# Autodesk Inventor assembly: Leg_joint_roll_pitch
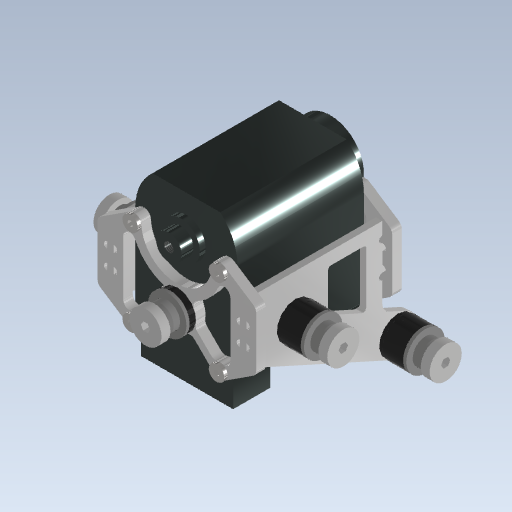
[picture p0: Inventor's stored thumbnail of the model, 512x512]
Saved by Autodesk Inventor 2020 (Build 240168000, 168)
## iProperties
Part Number: Leg_joint_roll_pitch
Document SubType Name: Assembly
Designer: Masato Kubotera
Mass: 155.537 g
Surface Area: 333.044 cm^2
Volume: 75.5065 cm^3
Density: 2.05992 g/cm^3
Author: Masato Kubotera
## Documents named in this file (16)
- C:\Users\Masato\Documents\Inventor\CIT Brains_Inventor\OpenPlatform_ver3_0 - Ver4_1branch\LowerBody\Leg_joit\Leg_joint_roll_pitch.iam
- C:\Users\Masato\Documents\Inventor\CIT Brains_Inventor\OpenPlatform_ver3_0 - Ver4_1branch\LowerBody\Leg_joit\Leg_joint_pitch_frame.ipt
- C:\Users\Masato\Documents\Inventor\CIT Brains_Inventor\OpenPlatform_ver3_0 - Ver4_1branch\LowerBody\Leg_joit\Leg_joint_roll_frame.ipt
- C:\Users\Masato\Documents\Inventor\CIT Brains_Inventor\OpenPlatform_ver3_0\Ready_Made\B3M11xx.ipt
- C:\Users\Masato\Documents\Inventor\CIT Brains_Inventor\OpenPlatform_ver3_0 - Ver4_1branch\Ready_Made\Screw\M2_6-20.ipt
- C:\Users\Masato\Documents\Inventor\CIT Brains_Inventor\OpenPlatform_ver3_0 - Ver4_1branch\Ready_Made\Screw\M2_6-15.ipt
- C:\Users\Masato\Documents\Inventor\CIT Brains_Inventor\OpenPlatform_ver3_0\Ready_Made\80F-0603.ipt
- C:\Users\Masato\Documents\Inventor\CIT Brains_Inventor\OpenPlatform_ver3_0\Ready_Made\CC-0612-15B.ipt
- C:\Users\Masato\Documents\Inventor\CIT Brains_Inventor\OpenPlatform_ver3_0\Ready_Made\CC-0612-50B.ipt
- C:\Users\Masato\Documents\Inventor\CIT Brains_Inventor\OpenPlatform_ver3_0 - Ver4_1branch\Ready_Made\SF419.ipt
- C:\Users\Masato\Documents\Inventor\CIT Brains_Inventor\OpenPlatform_ver3_0 - Ver4_1branch\Ready_Made\UUW-0412-10BH.ipt
- C:\Users\Masato\Documents\Inventor\CIT Brains_Inventor\OpenPlatform_ver3_0 - Ver4_1branch\Ready_Made\SLSBF6-39_5-M4-N4.ipt
- C:\Users\Masato\Documents\Inventor\CIT Brains_Inventor\OpenPlatform_ver3_0 - Ver4_1branch\Ready_Made\DBTS4-11-6.ipt
- C:\Users\Masato\Documents\Inventor\CIT Brains_Inventor\OpenPlatform_ver3_0 - Ver4_1branch\Ready_Made\DBS4-5-5.ipt
- C:\Users\Masato\Documents\Inventor\CIT Brains_Inventor\OpenPlatform_ver3_0 - Ver4_1branch\Ready_Made\DBTS4-10-4.ipt
- C:\Users\Masato\Documents\Inventor\CIT Brains_Inventor\OpenPlatform_ver3_0 - Ver4_1branch\Ready_Made\S4-07-3W.ipt
## Components (47 placed, 15 different names)
1. Leg_joint_pitch_frame:1 — フラッシュ:1, 挿入:192, 挿入:197, メイト:13
2. Leg_joint_pitch_frame:2 — フラッシュ:1, メイト:11, メイト:12, フラッシュ:7, 挿入:193, 挿入:194, 挿入:198
3. B3M11xx:1 — フラッシュ:6, メイト:8, メイト:10, 挿入:152, 挿入:153, 挿入:154, 挿入:155, 挿入:180, 挿入:181, 挿入:182, 挿入:183
4. M2_6-20:1 — 挿入:157
5. M2_6-20:2 — 挿入:159
6. M2_6-20:3 — 挿入:158
7. M2_6-20:4 — 挿入:160
8. M2_6-15:2 — 挿入:185
9. M2_6-15:3 — 挿入:186
10. 80F-0603:1 — 挿入:214
11. 80F-0603:3 — 挿入:130
12. 80F-0603:4 — 挿入:131
13. 80F-0603:5 — 挿入:129
14. 80F-0603:6 — 挿入:128
15. CC-0612-15B:1 — 挿入:114, 挿入:199
16. CC-0612-15B:2 — 挿入:115, 挿入:200
17. CC-0612-15B:3 — 挿入:116, 挿入:201
18. CC-0612-15B:4 — 挿入:117, 挿入:202
19. CC-0612-50B:1 — 挿入:114, 挿入:130
20. CC-0612-50B:2 — 挿入:115, 挿入:131
21. CC-0612-50B:3 — 挿入:116, 挿入:128
22. CC-0612-50B:4 — 挿入:117, 挿入:129
23. Leg_joint_roll_frame:1 — 挿入:152, 挿入:153, 挿入:154, 挿入:155, 挿入:157, 挿入:158, 挿入:159, 挿入:160, メイト:11, メイト:12, フラッシュ:7, 挿入:210, 挿入:217, 角度:2
24. 80F-0603:7 — 挿入:209
25. Leg_joint_roll_frame:2 — 挿入:180, 挿入:181, 挿入:182, 挿入:183, 挿入:185, 挿入:186, 挿入:207, 挿入:218, 角度:1
26. SF419:1 — 挿入:193, 挿入:195
27. SF419:2 — 挿入:192, 挿入:196
28. UUW-0412-10BH:1 — 挿入:194, 挿入:201, 挿入:203
29. UUW-0412-10BH:2 — 挿入:196, 挿入:199, 挿入:205
30. UUW-0412-10BH:3 — 挿入:195, 挿入:202, 挿入:204
31. UUW-0412-10BH:4 — 挿入:197, 挿入:200, 挿入:206
32. SLSBF6-39_5-M4-N4:1 — 挿入:198, メイト:13
33. DBTS4-11-6:1 — 挿入:203
34. DBTS4-11-6:2 — 挿入:206
35. DBTS4-11-6:3 — 挿入:204
36. DBTS4-11-6:4 — 挿入:205
37. UUW-0412-10BH:5 — 挿入:210, 挿入:213
38. UUW-0412-10BH:6 — 挿入:207, 挿入:208, 挿入:216
39. CC-0612-50B:5 — 挿入:208, 挿入:209
40. UUW-0412-10BH:7
41. UUW-0412-10BH:8
42. UUW-0412-10BH:9
43. UUW-0412-10BH:10 — 挿入:213, 挿入:214, 挿入:215
44. DBS4-5-5:1 — 挿入:215
45. DBTS4-10-4:1 — 挿入:216
46. S4-07-3W:1 — 挿入:217, 角度:2
47. S4-07-3W:2 — 挿入:218, 角度:1
## Relationships (57: Insert 47, Mate 5, Flush 3, Angle 2)
- フラッシュ:1 [Flush]: Leg_joint_pitch_frame:1 ↔ Leg_joint_pitch_frame:2
- フラッシュ:6 [Flush]: B3M11xx:1
- メイト:8 [Mate]: B3M11xx:1
- メイト:10 [Mate]: B3M11xx:1
- 挿入:114 [Insert]: CC-0612-15B:1 ↔ CC-0612-50B:1
- 挿入:115 [Insert]: CC-0612-15B:2 ↔ CC-0612-50B:2
- 挿入:116 [Insert]: CC-0612-15B:3 ↔ CC-0612-50B:3
- 挿入:117 [Insert]: CC-0612-15B:4 ↔ CC-0612-50B:4
- 挿入:128 [Insert]: 80F-0603:6 ↔ CC-0612-50B:3
- 挿入:129 [Insert]: 80F-0603:5 ↔ CC-0612-50B:4
- 挿入:130 [Insert]: 80F-0603:3 ↔ CC-0612-50B:1
- 挿入:131 [Insert]: 80F-0603:4 ↔ CC-0612-50B:2
- 挿入:152 [Insert]: B3M11xx:1 ↔ Leg_joint_roll_frame:1
- 挿入:153 [Insert]: B3M11xx:1 ↔ Leg_joint_roll_frame:1
- 挿入:154 [Insert]: B3M11xx:1 ↔ Leg_joint_roll_frame:1
- 挿入:155 [Insert]: B3M11xx:1 ↔ Leg_joint_roll_frame:1
- 挿入:157 [Insert]: M2_6-20:1 ↔ Leg_joint_roll_frame:1
- 挿入:158 [Insert]: M2_6-20:3 ↔ Leg_joint_roll_frame:1
- 挿入:159 [Insert]: M2_6-20:2 ↔ Leg_joint_roll_frame:1
- 挿入:160 [Insert]: M2_6-20:4 ↔ Leg_joint_roll_frame:1
- メイト:11 [Mate] (0.01 mm): Leg_joint_pitch_frame:2 ↔ Leg_joint_roll_frame:1
- メイト:12 [Mate] (0.01 mm): Leg_joint_pitch_frame:2 ↔ Leg_joint_roll_frame:1
- フラッシュ:7 [Flush]: Leg_joint_pitch_frame:2 ↔ Leg_joint_roll_frame:1
- 挿入:180 [Insert]: B3M11xx:1 ↔ Leg_joint_roll_frame:2
- 挿入:181 [Insert]: B3M11xx:1 ↔ Leg_joint_roll_frame:2
- 挿入:182 [Insert]: B3M11xx:1 ↔ Leg_joint_roll_frame:2
- 挿入:183 [Insert]: B3M11xx:1 ↔ Leg_joint_roll_frame:2
- 挿入:185 [Insert]: M2_6-15:2 ↔ Leg_joint_roll_frame:2
- 挿入:186 [Insert]: M2_6-15:3 ↔ Leg_joint_roll_frame:2
- 挿入:192 [Insert]: Leg_joint_pitch_frame:1 ↔ SF419:2
- 挿入:193 [Insert]: Leg_joint_pitch_frame:2 ↔ SF419:1
- 挿入:194 [Insert]: Leg_joint_pitch_frame:2 ↔ UUW-0412-10BH:1
- 挿入:195 [Insert]: SF419:1 ↔ UUW-0412-10BH:3
- 挿入:196 [Insert]: SF419:2 ↔ UUW-0412-10BH:2
- 挿入:197 [Insert]: Leg_joint_pitch_frame:1 ↔ UUW-0412-10BH:4
- 挿入:198 [Insert]: Leg_joint_pitch_frame:2 ↔ SLSBF6-39_5-M4-N4:1
- メイト:13 [Mate]: Leg_joint_pitch_frame:1 ↔ SLSBF6-39_5-M4-N4:1
- 挿入:199 [Insert]: CC-0612-15B:1 ↔ UUW-0412-10BH:2
- 挿入:200 [Insert]: CC-0612-15B:2 ↔ UUW-0412-10BH:4
- 挿入:201 [Insert]: CC-0612-15B:3 ↔ UUW-0412-10BH:1
- 挿入:202 [Insert]: CC-0612-15B:4 ↔ UUW-0412-10BH:3
- 挿入:203 [Insert]: UUW-0412-10BH:1 ↔ DBTS4-11-6:1
- 挿入:204 [Insert]: UUW-0412-10BH:3 ↔ DBTS4-11-6:3
- 挿入:205 [Insert]: UUW-0412-10BH:2 ↔ DBTS4-11-6:4
- 挿入:206 [Insert]: UUW-0412-10BH:4 ↔ DBTS4-11-6:2
- 挿入:207 [Insert]: Leg_joint_roll_frame:2 ↔ UUW-0412-10BH:6
- 挿入:208 [Insert]: UUW-0412-10BH:6 ↔ CC-0612-50B:5
- 挿入:209 [Insert]: 80F-0603:7 ↔ CC-0612-50B:5
- 挿入:210 [Insert]: Leg_joint_roll_frame:1 ↔ UUW-0412-10BH:5
- 挿入:213 [Insert]: UUW-0412-10BH:5 ↔ UUW-0412-10BH:10
- 挿入:214 [Insert]: 80F-0603:1 ↔ UUW-0412-10BH:10
- 挿入:215 [Insert]: UUW-0412-10BH:10 ↔ DBS4-5-5:1
- 挿入:216 [Insert]: UUW-0412-10BH:6 ↔ DBTS4-10-4:1
- 挿入:217 [Insert]: Leg_joint_roll_frame:1 ↔ S4-07-3W:1
- 挿入:218 [Insert]: Leg_joint_roll_frame:2 ↔ S4-07-3W:2
- 角度:1 [Angle] (0 deg): Leg_joint_roll_frame:2 ↔ S4-07-3W:2
- 角度:2 [Angle] (0 deg): Leg_joint_roll_frame:1 ↔ S4-07-3W:1
